# Autodesk Inventor assembly: FeeTechSTS3025BL
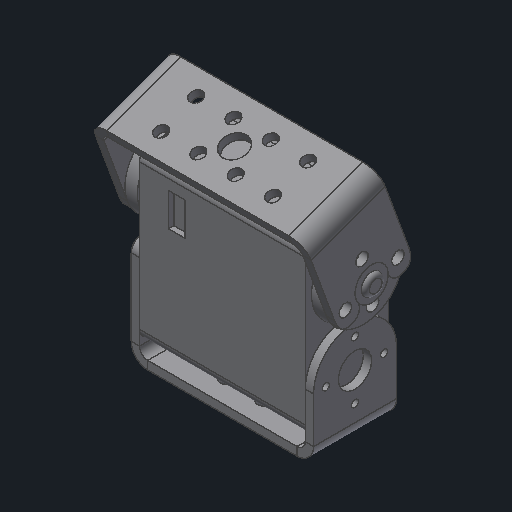
[picture p0: Inventor's stored thumbnail of the model, 512x512]
Saved by Autodesk Inventor 2025.2 (Build 292293000, 293)
## iProperties
Created: 2025-07-26
Part Number: FeeTechSTS3025BL
Document SubType Name: Assembly
Designer: valer
Author: valer
## Documents named in this file (5)
- C:\Users\valer\Desktop\str1ker\cad\external\NeckServo2\FeeTechSTS3025BL.iam
- C:\Users\valer\Desktop\str1ker\cad\external\NeckServo2\FeeTechSTS3025BL.ipt
- C:\Users\valer\Desktop\str1ker\cad\external\NeckServo2\FeeTechSTS3025BL-Flange.ipt
- C:\Users\valer\Desktop\str1ker\cad\external\NeckServo2\FeeTechSTS3025BL-BracketFixed.ipt
- C:\Users\valer\Desktop\str1ker\cad\external\NeckServo2\FeeTechSTS3025BL-BracketHorn.ipt
## Components (5 placed, 4 different names)
1. FeeTechSTS3025BL:1 — Mate:1, Mate:2, Mate:3, Mate:4, Flush:6, Flush:1, Flush:7, Flush:8, Mate:8, Mate:9, Mate:10
2. FeeTechSTS3025BL-Flange:1 — Mate:1, Mate:2
3. FeeTechSTS3025BL-Flange:2 — Mate:3, Mate:4, Flush:9, Mate:5, Mate:6, Mate:7
4. FeeTechSTS3025BL-BracketFixed:1 — Flush:8, Mate:8, Mate:9, Mate:10
5. FeeTechSTS3025BL-BracketHorn:1 — Flush:9, Mate:5, Mate:6, Mate:7
## Relationships (15: Mate 10, Flush 5)
- Mate:1: FeeTechSTS3025BL:1 ↔ FeeTechSTS3025BL-Flange:1
- Mate:2: FeeTechSTS3025BL:1 ↔ FeeTechSTS3025BL-Flange:1
- Mate:3: FeeTechSTS3025BL:1 ↔ FeeTechSTS3025BL-Flange:2
- Mate:4: FeeTechSTS3025BL:1 ↔ FeeTechSTS3025BL-Flange:2
- Flush:6: FeeTechSTS3025BL:1
- Flush:1: FeeTechSTS3025BL:1
- Flush:7: FeeTechSTS3025BL:1
- Flush:8: FeeTechSTS3025BL:1 ↔ FeeTechSTS3025BL-BracketFixed:1
- Flush:9: FeeTechSTS3025BL-Flange:2 ↔ FeeTechSTS3025BL-BracketHorn:1
- Mate:5: FeeTechSTS3025BL-Flange:2 ↔ FeeTechSTS3025BL-BracketHorn:1
- Mate:6: FeeTechSTS3025BL-Flange:2 ↔ FeeTechSTS3025BL-BracketHorn:1
- Mate:7: FeeTechSTS3025BL-Flange:2 ↔ FeeTechSTS3025BL-BracketHorn:1
- Mate:8: FeeTechSTS3025BL:1 ↔ FeeTechSTS3025BL-BracketFixed:1
- Mate:9: FeeTechSTS3025BL:1 ↔ FeeTechSTS3025BL-BracketFixed:1
- Mate:10: FeeTechSTS3025BL:1 ↔ FeeTechSTS3025BL-BracketFixed:1
